# Autodesk Inventor assembly: Сборка1
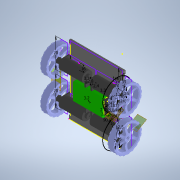
[picture p0: Inventor's stored thumbnail of the model, 180x180]
Saved by Autodesk Inventor 2020 (Build 240168000, 168)
## iProperties
Created: 2022-07-15
Part Number: Сборка1
Document SubType Name: Assembly
Designer: akapu
Author: akapu
## Documents named in this file (10)
- C:\Users\akapu\Documents\maze bot\Сборка1.iam
- C:\Users\akapu\Documents\maze bot\maze_02.ipt
- C:\Users\akapu\Documents\maze bot\battery pack_1.ipt
- C:\Users\akapu\Documents\maze bot\battery_2.1.ipt
- C:\Users\akapu\Documents\maze bot\battery_2.2.ipt
- C:\Users\akapu\Documents\maze bot\motor.ipt
- C:\Users\akapu\Documents\maze bot\motor_ЗЕРКАЛО2.ipt
- C:\Users\akapu\Documents\maze bot\motor_ЗЕРКАЛО3.ipt
- C:\Users\akapu\Documents\maze bot\motor_ЗЕРКАЛО2_ЗЕРКАЛО.ipt
- C:\Users\akapu\Documents\maze bot\wheel.ipt
## Components (12 placed, 9 different names)
1. maze_02:1 — Вставка:1, Вставка:2, Совмещение:2, Совмещение:3, Совмещение:4, Совмещение:5
2. battery_2.1:1 — Вставка:1
3. battery_2.2:1 — Вставка:2, Совмещение:6
4. motor:1 — Совмещение:5, С поворотом:2
5. motor_ЗЕРКАЛО2:1 — Совмещение:4, С поворотом:1
6. motor_ЗЕРКАЛО3:1 — Совмещение:2, С поворотом:3
7. motor_ЗЕРКАЛО2_ЗЕРКАЛО:1 — Совмещение:3, С поворотом:4
8. battery pack_1:2 — Совмещение:6
9. wheel:1 — С поворотом:1
10. wheel:2 — С поворотом:2
11. wheel:3 — С поворотом:3
12. wheel:4 — С поворотом:4
## Relationships (11: Mate 5, RevoluteJoint 4, Insert 2)
- Вставка:1 [Insert]: maze_02:1 ↔ battery_2.1:1
- Вставка:2 [Insert]: maze_02:1 ↔ battery_2.2:1
- Совмещение:2 [Mate]: maze_02:1 ↔ motor_ЗЕРКАЛО3:1
- Совмещение:3 [Mate]: maze_02:1 ↔ motor_ЗЕРКАЛО2_ЗЕРКАЛО:1
- Совмещение:4 [Mate]: maze_02:1 ↔ motor_ЗЕРКАЛО2:1
- Совмещение:5 [Mate]: maze_02:1 ↔ motor:1
- Совмещение:6 [Mate]: battery_2.2:1 ↔ battery pack_1:2
- С поворотом:1 [RevoluteJoint] (5 mm): motor_ЗЕРКАЛО2:1 ↔ wheel:1
- С поворотом:2 [RevoluteJoint]: motor:1 ↔ wheel:2
- С поворотом:3 [RevoluteJoint] (5 mm): motor_ЗЕРКАЛО3:1 ↔ wheel:3
- С поворотом:4 [RevoluteJoint]: motor_ЗЕРКАЛО2_ЗЕРКАЛО:1 ↔ wheel:4
